# Autodesk Inventor assembly: CuboidSecurityBoxOpenedLayer
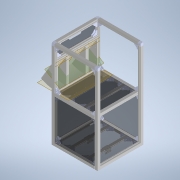
[picture p0: Inventor's stored thumbnail of the model, 180x180]
Saved by Autodesk Inventor 2021.3 (Build 253353000, 353)
## iProperties
Created: 2020-11-09
Part Number: CuboidSecurityBoxOpenedLayer
Document SubType Name: Assembly
Designer: gisen
Author: gisen
## Documents named in this file (3)
- C:\Users\gisen\GitProjects\CAD-Data\CuboidAccessories\SecurityBox\CuboidSecurityBoxOpenedLayer.iam
- C:\Users\gisen\GitProjects\CAD-Data\CuboidAccessories\SecurityBox\Assemblies\CuboidSecurityBoxBasisTypeB.iam
- C:\Users\gisen\GitProjects\CAD-Data\CuboidAccessories\SecurityBox\Assemblies\AdditionalLayerAssembly.iam
## Components (2 placed, 2 different names)
1. CuboidSecurityBoxBasisTypeB:1 [sub-assembly] — フラッシュ:1, メイト:1, フラッシュ:2, フラッシュ:3, フラッシュ:4, フラッシュ:5
2. AdditionalLayerAssembly:1 [sub-assembly] — フラッシュ:1, メイト:1, フラッシュ:2
## Relationships (6: Flush 5, Mate 1)
- フラッシュ:1 [Flush] (20 mm): CuboidSecurityBoxBasisTypeB:1 ↔ AdditionalLayerAssembly:1
- メイト:1 [Mate]: CuboidSecurityBoxBasisTypeB:1 ↔ AdditionalLayerAssembly:1
- フラッシュ:2 [Flush]: CuboidSecurityBoxBasisTypeB:1 ↔ AdditionalLayerAssembly:1
- フラッシュ:3 [Flush]: CuboidSecurityBoxBasisTypeB:1
- フラッシュ:4 [Flush]: CuboidSecurityBoxBasisTypeB:1
- フラッシュ:5 [Flush]: CuboidSecurityBoxBasisTypeB:1
